# Autodesk Inventor assembly: ASM Printing Head
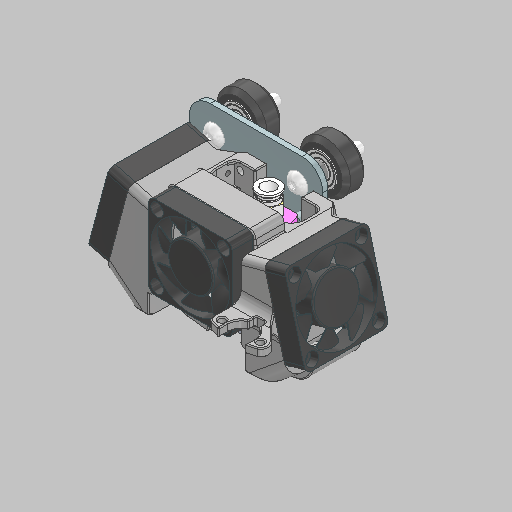
[picture p0: Inventor's stored thumbnail of the model, 512x512]
Saved by Autodesk Inventor 2025.4 (Build 294407000, 407)
## iProperties
Created: 2026-03-02
Part Number: ASM Printing Head
Document SubType Name: Assembly
Designer: Inema
Author: Inema
Revision Number: ANY
## Documents named in this file (8)
- C:\Users\Inema\OneDrive\GitHub\Ender-3\Ender-3 Mechanical\Modificada\Extrusor Original\ASM Printing Head.iam
- C:\Users\Inema\OneDrive\GitHub\Ender-3\Ender-3 Mechanical\Modificada\E plate.ipt
- C:\Users\Inema\OneDrive\GitHub\Ender-3\Ender-3 Mechanical\Modificada\Nozzle fan.ipt
- C:\Users\Inema\OneDrive\GitHub\Ender-3\Ender-3 Mechanical\Modificada\ASM Heating Unit.iam
- C:\Users\Inema\OneDrive\GitHub\Ender-3\Ender-3 Mechanical\Modificada\ASM Roller X-Axis.iam
- C:\Users\Inema\OneDrive\GitHub\Ender-3\Ender-3 Mechanical\Modificada\ASM Eccentrical Roller X-Axis.iam
- C:\Users\Inema\OneDrive\GitHub\Ender-3\Ender-3 Mechanical\Modificada\M3X6Pan Head Screw.ipt
- C:\Users\Inema\OneDrive\GitHub\Ender-3\Ender-3 Mechanical\Modificada\mS_Ender_Dual_4010_1.1\mS_Ender_Dual_4010_1.1.ipt
## Components (11 placed, 10 different names)
1. E plate_168 — Ángulo:1, Coincidencia:6, Coincidencia:7, Coincidencia:9, Coincidencia:10
2. Nozzle fan_172 — Coincidencia:16, Coincidencia:17, Coincidencia:18
3. ASM Heating Unit_173 [sub-assembly] — Ángulo:1, Coincidencia:6, Coincidencia:7, Coincidencia:11, Coincidencia:12
4. ASM Roller X-Axis_174 [sub-assembly]
5. ASM Roller X-Axis_175 [sub-assembly]
6. ASM Eccentrical Roller X-Axis_176 [sub-assembly]
7. M3X6Pan Head Screw_182
8. M3X6Pan Head Screw_183 — Coincidencia:9
9. Nozzle fan:2 — Coincidencia:13, Coincidencia:14, Coincidencia:15
10. mS_Ender_Dual_4010_1.1:1 — Coincidencia:10, Coincidencia:11, Coincidencia:12, Coincidencia:13, Coincidencia:14, Coincidencia:15, Coincidencia:16, Coincidencia:17, Coincidencia:18, Coincidencia:19, Coincidencia:20, Coincidencia:21
11. Nozzle fan:3 — Coincidencia:19, Coincidencia:20, Coincidencia:21
## Relationships (16: Mate 15, Angle 1)
- Ángulo:1 [Angle] (0 deg): E plate_168 ↔ ASM Heating Unit_173
- Coincidencia:6 [Mate]: E plate_168 ↔ ASM Heating Unit_173
- Coincidencia:7 [Mate]: E plate_168 ↔ ASM Heating Unit_173
- Coincidencia:9 [Mate]: E plate_168 ↔ M3X6Pan Head Screw_183
- Coincidencia:10 [Mate]: E plate_168 ↔ mS_Ender_Dual_4010_1.1:1
- Coincidencia:11 [Mate] (11 mm): ASM Heating Unit_173 ↔ mS_Ender_Dual_4010_1.1:1
- Coincidencia:12 [Mate] (-1 mm): ASM Heating Unit_173 ↔ mS_Ender_Dual_4010_1.1:1
- Coincidencia:13 [Mate]: Nozzle fan:2 ↔ mS_Ender_Dual_4010_1.1:1
- Coincidencia:14 [Mate]: Nozzle fan:2 ↔ mS_Ender_Dual_4010_1.1:1
- Coincidencia:15 [Mate]: Nozzle fan:2 ↔ mS_Ender_Dual_4010_1.1:1
- Coincidencia:16 [Mate]: Nozzle fan_172 ↔ mS_Ender_Dual_4010_1.1:1
- Coincidencia:17 [Mate]: Nozzle fan_172 ↔ mS_Ender_Dual_4010_1.1:1
- Coincidencia:18 [Mate]: Nozzle fan_172 ↔ mS_Ender_Dual_4010_1.1:1
- Coincidencia:19 [Mate]: mS_Ender_Dual_4010_1.1:1 ↔ Nozzle fan:3
- Coincidencia:20 [Mate]: mS_Ender_Dual_4010_1.1:1 ↔ Nozzle fan:3
- Coincidencia:21 [Mate]: mS_Ender_Dual_4010_1.1:1 ↔ Nozzle fan:3
